# Autodesk Inventor assembly: KB33-046-008 - Блок АКБ
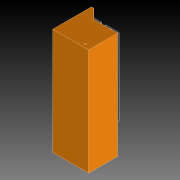
[picture p0: Inventor's stored thumbnail of the model, 180x180]
Saved by Autodesk Inventor 2020 (Build 240168000, 168)
## iProperties
Created: 2021-08-09
Part Number: KB33-046-008 - Блок АКБ
Document SubType Name: Assembly
Designer: Петров Иван
Mass: 907.498 g
Surface Area: 1539.1 cm^2
Volume: 907.498 cm^3
Density: 1 g/cm^3
Author: Петров Иван
## Documents named in this file (3)
- E:\IVAN\Ivan_desktop\Kvantorium\Projects\RoboPatrol\design\KB33-046-008 - Блок АКБ.iam
- E:\IVAN\Ivan_desktop\Kvantorium\Projects\RoboPatrol\design\KB33-046-008-001 - Корпус.ipt
- E:\IVAN\Ivan_desktop\Kvantorium\Projects\RoboPatrol\design\standart_components\Turnigy 4S 5200 mah\Turnigy 4S 5200 mah.ipt
## Components (3 placed, 2 different names)
1. KB33-046-008-001 - Корпус:1 — Совмещение:2, Совмещение:3, Совмещение:4, Совмещение:5, Совмещение:6
2. Turnigy 4S 5200 mah:1 — Совмещение:2, Совмещение:3, Совмещение:4, Заподлицо:1
3. Turnigy 4S 5200 mah:2 — Совмещение:5, Заподлицо:1, Совмещение:6
## Relationships (6: Mate 5, Flush 1)
- Совмещение:2 [Mate]: KB33-046-008-001 - Корпус:1 ↔ Turnigy 4S 5200 mah:1
- Совмещение:3 [Mate]: KB33-046-008-001 - Корпус:1 ↔ Turnigy 4S 5200 mah:1
- Совмещение:4 [Mate]: KB33-046-008-001 - Корпус:1 ↔ Turnigy 4S 5200 mah:1
- Совмещение:5 [Mate]: KB33-046-008-001 - Корпус:1 ↔ Turnigy 4S 5200 mah:2
- Заподлицо:1 [Flush]: Turnigy 4S 5200 mah:1 ↔ Turnigy 4S 5200 mah:2
- Совмещение:6 [Mate]: KB33-046-008-001 - Корпус:1 ↔ Turnigy 4S 5200 mah:2
